# Autodesk Inventor assembly: Series Elastic Gearbox
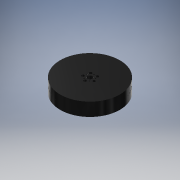
[picture p0: Inventor's stored thumbnail of the model, 180x180]
Saved by Autodesk Inventor 2017 (Build 210142000, 142)
## iProperties
Created: 2019-09-21
Part Number: Series Elastic Gearbox
Document SubType Name: Assembly
Designer: Dell
Author: Dell
## Documents named in this file (3)
- C:\Users\Dell\Documents\GitHub\tr2\Actuator 1.6\Series Elastic Gearbox\Series Elastic Gearbox.iam
- C:\Users\Dell\Documents\GitHub\tr2\Actuator 1.6\Series Elastic Gearbox\SG01.ipt
- C:\Users\Dell\Documents\GitHub\tr2\Actuator 1.6\Series Elastic Gearbox\SG02.ipt
## Components (2 placed, 2 different names)
1. SG01:1 — Mate:1, Mate:2
2. SG02:1 — Mate:1, Mate:2
## Relationships (2: Mate 2)
- Mate:1: SG01:1 ↔ SG02:1
- Mate:2: SG01:1 ↔ SG02:1
